# Autodesk Inventor assembly: NFC_module
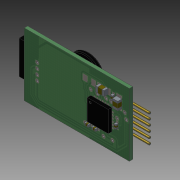
[picture p0: Inventor's stored thumbnail of the model, 180x180]
Saved by Autodesk Inventor 2013 (Build 170138000, 138)
## iProperties
Created: 2015-07-04
Part Number: NFC_module
Document SubType Name: Assembly
Designer: terg
Author: terg
## Documents named in this file (9)
- C:\Users\terg\Projects\ModularElectronics\3D_models\NFC_module\NFC_module.iam
- C:\Users\terg\Projects\ModularElectronics\3D_models\NFC_module\NFC_module_PCB.ipt
- C:\Users\terg\Projects\ModularElectronics\3D_models\Components\0805_cap.ipt
- C:\Users\terg\Projects\ModularElectronics\3D_models\Components\0402_cap.ipt
- C:\Users\terg\Projects\ModularElectronics\3D_models\Components\EFM32ZG110.ipt
- C:\Users\terg\Projects\ModularElectronics\3D_models\NFC_module\AS3953.ipt
- C:\Users\terg\Projects\ModularElectronics\3D_models\NFC_module\PA6512.ipt
- C:\Users\terg\Projects\ModularElectronics\3D_models\Components\FemalConnector.ipt
- C:\Users\terg\Projects\ModularElectronics\3D_models\Components\MaleConnector.ipt
## Components (14 placed, 8 different names)
1. NFC_module_PCB:1 — Zestawiający:1, Zestawiający:2, Zestawiający:3, Zestawiający:4, Zestawiający:5, Zestawiający:7, Równoległy:1, Równoległy:2, Równoległy:3, Równoległy:4, Równoległy:5, Równoległy:6, Równoległy:7, Równoległy:8, Równoległy:9, Równoległy:10, Równoległy:11, Równoległy:12, Zestawiający:8, Równoległy:13, Równoległy:14, Zestawiający:9, Zestawiający:10, Równoległy:15, Równoległy:16, Równoległy:17, Równoległy:18, Zestawiający:11, Równoległy:19, Równoległy:20, Zestawiający:12, Równoległy:21, Równoległy:22, Zestawiający:13, Zestawiający:14, Równoległy:23, Równoległy:24, Równoległy:25, Równoległy:26
2. 0805_cap:1 — Zestawiający:1, Równoległy:1, Równoległy:2
3. 0805_cap:2 — Zestawiający:2, Równoległy:4, Równoległy:5
4. 0402_cap:1 — Zestawiający:3, Równoległy:7, Równoległy:8
5. 0402_cap:2 — Zestawiający:4, Równoległy:9, Równoległy:10
6. 0402_cap:3 — Zestawiający:5, Równoległy:11, Równoległy:12
7. 0402_cap:5 — Zestawiający:7, Równoległy:3, Równoległy:6
8. EFM32ZG110:1 — Zestawiający:8, Równoległy:13, Równoległy:14
9. 0402_cap:6 — Zestawiający:9, Równoległy:15, Równoległy:17
10. 0805_cap:3 — Zestawiający:10, Równoległy:16, Równoległy:18
11. AS3953:1 — Zestawiający:11, Równoległy:19, Równoległy:20
12. PA6512:1 — Zestawiający:12, Równoległy:21, Równoległy:22
13. FemalConnector:1 — Zestawiający:13, Równoległy:23, Równoległy:24
14. MaleConnector:1 — Zestawiający:14, Równoległy:25, Równoległy:26
## Relationships (39: Flush 26, Mate 13)
- Zestawiający:1 [Mate]: NFC_module_PCB:1 ↔ 0805_cap:1
- Zestawiający:2 [Mate]: NFC_module_PCB:1 ↔ 0805_cap:2
- Zestawiający:3 [Mate]: NFC_module_PCB:1 ↔ 0402_cap:1
- Zestawiający:4 [Mate]: NFC_module_PCB:1 ↔ 0402_cap:2
- Zestawiający:5 [Mate]: NFC_module_PCB:1 ↔ 0402_cap:3
- Zestawiający:7 [Mate]: NFC_module_PCB:1 ↔ 0402_cap:5
- Równoległy:1 [Flush] (5.044 mm): NFC_module_PCB:1 ↔ 0805_cap:1
- Równoległy:2 [Flush] (2.464 mm): NFC_module_PCB:1 ↔ 0805_cap:1
- Równoległy:3 [Flush] (3.01 mm): NFC_module_PCB:1 ↔ 0402_cap:5
- Równoległy:4 [Flush] (3.044 mm): NFC_module_PCB:1 ↔ 0805_cap:2
- Równoległy:5 [Flush] (1.785 mm): NFC_module_PCB:1 ↔ 0805_cap:2
- Równoległy:6 [Flush] (3.475 mm): NFC_module_PCB:1 ↔ 0402_cap:5
- Równoległy:7 [Flush] (2.645 mm): NFC_module_PCB:1 ↔ 0402_cap:1
- Równoległy:8 [Flush] (8.527 mm): NFC_module_PCB:1 ↔ 0402_cap:1
- Równoległy:9 [Flush] (7.494 mm): NFC_module_PCB:1 ↔ 0402_cap:2
- Równoległy:10 [Flush] (11.877 mm): NFC_module_PCB:1 ↔ 0402_cap:2
- Równoległy:11 [Flush] (11.856 mm): NFC_module_PCB:1 ↔ 0402_cap:3
- Równoległy:12 [Flush] (9.19 mm): NFC_module_PCB:1 ↔ 0402_cap:3
- Zestawiający:8 [Mate]: NFC_module_PCB:1 ↔ EFM32ZG110:1
- Równoległy:13 [Flush] (5.981 mm): NFC_module_PCB:1 ↔ EFM32ZG110:1
- Równoległy:14 [Flush] (4.166 mm): NFC_module_PCB:1 ↔ EFM32ZG110:1
- Zestawiający:9 [Mate]: NFC_module_PCB:1 ↔ 0402_cap:6
- Zestawiający:10 [Mate]: NFC_module_PCB:1 ↔ 0805_cap:3
- Równoległy:15 [Flush] (8.278 mm): NFC_module_PCB:1 ↔ 0402_cap:6
- Równoległy:16 [Flush] (7.176 mm): NFC_module_PCB:1 ↔ 0805_cap:3
- Równoległy:17 [Flush] (9.044 mm): NFC_module_PCB:1 ↔ 0402_cap:6
- Równoległy:18 [Flush] (9.967 mm): NFC_module_PCB:1 ↔ 0805_cap:3
- Zestawiający:11 [Mate]: NFC_module_PCB:1 ↔ AS3953:1
- Równoległy:19 [Flush] (6.041 mm): NFC_module_PCB:1 ↔ AS3953:1
- Równoległy:20 [Flush] (6.5 mm): NFC_module_PCB:1 ↔ AS3953:1
- Zestawiający:12 [Mate]: NFC_module_PCB:1 ↔ PA6512:1
- Równoległy:21 [Flush] (1.075 mm): NFC_module_PCB:1 ↔ PA6512:1
- Równoległy:22 [Flush] (4.545 mm): NFC_module_PCB:1 ↔ PA6512:1
- Zestawiający:13 [Mate]: NFC_module_PCB:1 ↔ FemalConnector:1
- Zestawiający:14 [Mate]: NFC_module_PCB:1 ↔ MaleConnector:1
- Równoległy:23 [Flush] (3.547 mm): NFC_module_PCB:1 ↔ FemalConnector:1
- Równoległy:24 [Flush] (-2.042 mm): NFC_module_PCB:1 ↔ FemalConnector:1
- Równoległy:25 [Flush] (-3.287 mm): NFC_module_PCB:1 ↔ MaleConnector:1
- Równoległy:26 [Flush] (-4.079 mm): NFC_module_PCB:1 ↔ MaleConnector:1
